# Autodesk Inventor assembly: roofPanel3
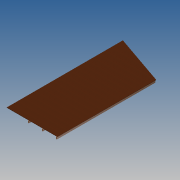
[picture p0: Inventor's stored thumbnail of the model, 180x180]
Saved by Autodesk Inventor 2013 (Build 170138000, 138)
## iProperties
Created: 2013-08-10
Part Number: roofPanel3
Document SubType Name: Assembly
Designer: ddeboer
Author: ddeboer
## Documents named in this file (3)
- C:\Users\ddeboer\Desktop\porch\roofPanel3.iam
- C:\Users\ddeboer\Desktop\porch\2by4cross.ipt
- C:\Users\ddeboer\Desktop\porch\roof2.ipt
## Components (4 placed, 2 different names)
1. roof2:1 — Mate:1
2. 2by4cross:1 — Mate:1
3. 2by4cross:2
4. 2by4cross:3
## Component patterns: (3 elements, first: 2by4cross:1)
## Relationships (1: Mate 1)
- Mate:1: roof2:1 ↔ 2by4cross:1
